# Autodesk Inventor assembly: DribblerUnit
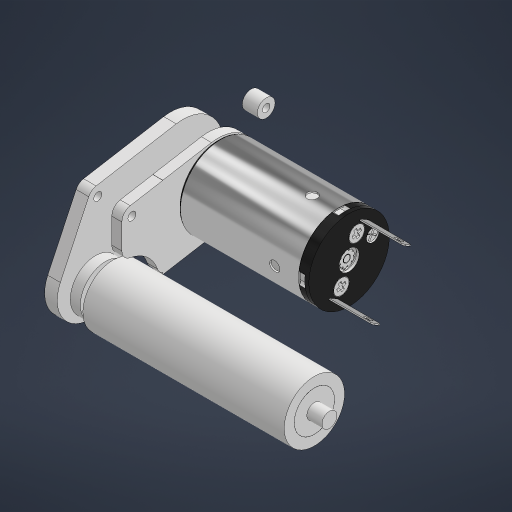
[picture p0: Inventor's stored thumbnail of the model, 512x512]
Saved by Autodesk Inventor 2024.2 (Build 282272000, 272)
## iProperties
Created: 2023-12-27
Part Number: DribblerUnit
Document SubType Name: Assembly
Designer: Hanaoka
Author: Hanaoka
## Documents named in this file (11)
- G:\共有ドライブ\reRo\05_個人\hanaoka\inventor\DribblerUnit\DribblerUnit.iam
- G:\共有ドライブ\reRo\05_個人\hanaoka\inventor\DribblerUnit\Dribbler_Tube.ipt
- G:\共有ドライブ\reRo\05_個人\hanaoka\inventor\DribblerUnit\Shaft_350.ipt
- G:\共有ドライブ\reRo\05_個人\hanaoka\inventor\DribblerUnit\Bearing_C-FL673ZZ\Bearing_C-FL673ZZ.ipt
- G:\共有ドライブ\reRo\05_個人\hanaoka\inventor\DribblerUnit\Tube_Hub.ipt
- G:\共有ドライブ\reRo\05_個人\hanaoka\inventor\DribblerUnit\Althonix16dct\Althonix16dct.ipt
- G:\共有ドライブ\reRo\05_個人\hanaoka\inventor\HandleUnit\MotorMount.ipt
- G:\共有ドライブ\reRo\05_個人\hanaoka\inventor\HandleUnit\GearCover.ipt
- G:\共有ドライブ\reRo\05_個人\hanaoka\inventor\HandleUnit\Pinion_Gear.ipt
- G:\共有ドライブ\reRo\05_個人\hanaoka\inventor\HandleUnit\OutSide_Gear.ipt
- G:\共有ドライブ\reRo\05_個人\hanaoka\inventor\Pinion_9T0.4M.ipt
## Components (10 placed, 10 different names)
1. Dribbler_Tube:1 — 挿入:2
2. Shaft_350:1 — 挿入:1, 挿入:4, 挿入:8
3. Bearing_C-FL673ZZ:1 — 挿入:1, 挿入:6
4. Tube_Hub:1 — 挿入:2, 挿入:4
5. Althonix16dct:1 — 挿入:5, メイト:1, 挿入:7
6. MotorMount:1 — 挿入:5, メイト:1
7. GearCover:1 — 挿入:6
8. Pinion_Gear:1 — 挿入:7
9. OutSide_Gear:1 — 挿入:8
10. Pinion_9T0.4M:1
## Relationships (8: Insert 7, Mate 1)
- 挿入:1 [Insert]: Shaft_350:1 ↔ Bearing_C-FL673ZZ:1
- 挿入:2 [Insert]: Dribbler_Tube:1 ↔ Tube_Hub:1
- 挿入:4 [Insert] (12 mm): Shaft_350:1 ↔ Tube_Hub:1
- 挿入:5 [Insert]: Althonix16dct:1 ↔ MotorMount:1
- メイト:1 [Mate]: Althonix16dct:1 ↔ MotorMount:1
- 挿入:6 [Insert]: Bearing_C-FL673ZZ:1 ↔ GearCover:1
- 挿入:7 [Insert] (2.5 mm): Althonix16dct:1 ↔ Pinion_Gear:1
- 挿入:8 [Insert] (3.5 mm): Shaft_350:1 ↔ OutSide_Gear:1
